# Autodesk Inventor assembly: Assembly
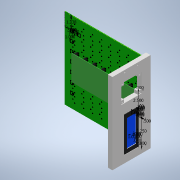
[picture p0: Inventor's stored thumbnail of the model, 180x180]
Saved by Autodesk Inventor 2020 (Build 240168000, 168)
## iProperties
Created: 2019-12-03
Part Number: Assembly
Document SubType Name: Assembly
Designer: torto
Author: torto
## Documents named in this file (7)
- C:\Users\torto\OneDrive\Documents\Projects\LED Cube\Mechanical\Inventor\CubeAssembly.iam
- C:\Users\torto\OneDrive\Documents\Projects\LED Cube\Mechanical\Inventor\Cube_Pcb.ipt
- C:\Users\torto\OneDrive\Documents\Projects\LED Cube\Mechanical\Inventor\CubeBase.ipt
- C:\Users\torto\OneDrive\Documents\Projects\LED Cube\Mechanical\Inventor\CubeBaseFront.ipt
- C:\Users\torto\OneDrive\Documents\Projects\LED Cube\Mechanical\Inventor\LcdAssembly.ipt
- C:\Users\torto\OneDrive\Documents\Projects\LED Cube\Mechanical\Inventor\1x8 SMD Header.ipt
- C:\Users\torto\OneDrive\Documents\Projects\LED Cube\Mechanical\Inventor\DaughterBoard.ipt
## Components (31 placed, 8 different names)
1. RearPanel — Flush:1, Flush:2, Mate:1, Flush:3, Flush:4, Mate:2, Mate:3, Mate:4
2. RightPanel — Flush:1, Flush:2, Mate:1
3. CubeBase:3 — Flush:3, Flush:4, Mate:2, Mate:5, Mate:6, Flush:5, Flush:6
4. BasePcb — Mate:3, Mate:4, Mate:5, Mate:10, Mate:11, Mate:12
5. FrontPanel — Mate:6, Flush:5, Flush:6, Mate:7, Mate:8, Mate:9
6. LcdAssembly:1 — Mate:7, Mate:8, Mate:9
7. DaughterBoard:1 — Mate:13, Flush:7, Flush:8
8. 1x8 SMD Header:1 — Mate:10, Mate:11, Mate:12, Flush:7, Flush:8
9. 1x8 SMD Header:2
10. 1x8 SMD Header:3
11. 1x8 SMD Header:4
12. 1x8 SMD Header:5
13. 1x8 SMD Header:6
14. 1x8 SMD Header:7
15. 1x8 SMD Header:8 — Mate:13
16. 1x8 SMD Header:9
17. 1x8 SMD Header:10
18. 1x8 SMD Header:11
19. 1x8 SMD Header:12
20. 1x8 SMD Header:13
21. 1x8 SMD Header:14
22. 1x8 SMD Header:15
23. 1x8 SMD Header:16
24. 1x8 SMD Header:17
25. 1x8 SMD Header:18
26. 1x8 SMD Header:19
27. 1x8 SMD Header:20
28. 1x8 SMD Header:21
29. 1x8 SMD Header:22
30. 1x8 SMD Header:23
31. 1x8 SMD Header:24
## Component patterns: (24 elements, first: 1x8 SMD Header:1)
## Relationships (21: Mate 13, Flush 8)
- Flush:1: RearPanel ↔ RightPanel
- Flush:2: RearPanel ↔ RightPanel
- Mate:1: RearPanel ↔ RightPanel
- Flush:3: RearPanel ↔ CubeBase:3
- Flush:4: RearPanel ↔ CubeBase:3
- Mate:2: RearPanel ↔ CubeBase:3
- Mate:3: RearPanel ↔ BasePcb
- Mate:4: RearPanel ↔ BasePcb
- Mate:5: CubeBase:3 ↔ BasePcb
- Mate:6: CubeBase:3 ↔ FrontPanel
- Flush:5: CubeBase:3 ↔ FrontPanel
- Flush:6: CubeBase:3 ↔ FrontPanel
- Mate:7: FrontPanel ↔ LcdAssembly:1
- Mate:8: FrontPanel ↔ LcdAssembly:1
- Mate:9: FrontPanel ↔ LcdAssembly:1
- Mate:10: BasePcb ↔ 1x8 SMD Header:1
- Mate:11: BasePcb ↔ 1x8 SMD Header:1
- Mate:12: BasePcb ↔ 1x8 SMD Header:1
- Mate:13: DaughterBoard:1 ↔ 1x8 SMD Header:8
- Flush:7: DaughterBoard:1 ↔ 1x8 SMD Header:1
- Flush:8: DaughterBoard:1 ↔ 1x8 SMD Header:1
